# Autodesk Inventor assembly: ScimitarPropellerModel1
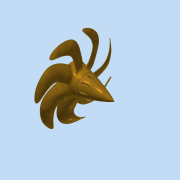
[picture p0: Inventor's stored thumbnail of the model, 180x180]
Saved by Autodesk Inventor 2017.3 (Build 213256000, 256)
## iProperties
Created: 2018-06-17
Part Number: ScimitarPropellerModel1
Document SubType Name: Assembly
Designer: Derek Wider
Author: Derek Wider
## Documents named in this file (3)
- G:\Projects\Submarine\Submarine-project\CAD\Downloaded\ScimitarProp\ScimitarPropellerModel1.iam
- G:\Projects\Submarine\Submarine-project\CAD\Downloaded\ScimitarProp\ScimitarPropellerBase1.ipt
- G:\Projects\Submarine\Submarine-project\CAD\Downloaded\ScimitarProp\ScimitarPropellerCap1.ipt
## Components (2 placed, 2 different names)
1. ScimitarPropellerBase1:1 — Mate:1, Mate:2
2. ScimitarPropellerCap1:1 — Mate:1, Mate:2
## Relationships (2: Mate 2)
- Mate:1: ScimitarPropellerBase1:1 ↔ ScimitarPropellerCap1:1
- Mate:2: ScimitarPropellerBase1:1 ↔ ScimitarPropellerCap1:1
